# Autodesk Inventor assembly: Case
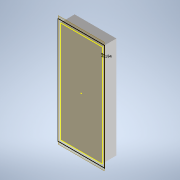
[picture p0: Inventor's stored thumbnail of the model, 180x180]
Saved by Autodesk Inventor 2020 (Build 240168000, 168)
## iProperties
Created: 2019-12-17
Part Number: Case
Document SubType Name: Assembly
Designer: erwin
Author: erwin
## Documents named in this file (4)
- D:\GitHub\ElCheapoAIS-nmea\case\Wooden Multicase\Case.iam
- D:\GitHub\ElCheapoAIS-nmea\case\Wooden Multicase\interior.ipt
- D:\GitHub\ElCheapoAIS-nmea\case\Wooden Multicase\cover.ipt
- D:\GitHub\ElCheapoAIS-nmea\case\Wooden Multicase\parameters.ipt
## Components (3 placed, 3 different names)
1. interior:1 — Flush:1, Flush:2
2. cover:1 — Flush:1, Flush:2
3. parameters:1
## Relationships (2: Flush 2)
- Flush:1: interior:1 ↔ cover:1
- Flush:2: interior:1 ↔ cover:1
